# Autodesk Inventor assembly: Gantry Table With Chucks - V2
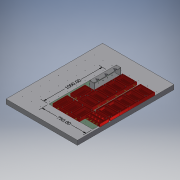
[picture p0: Inventor's stored thumbnail of the model, 180x180]
Saved by Autodesk Inventor 2019.4 (Build 234330000, 330)
## iProperties
Created: 2021-03-04
Part Number: Gantry Table With Chucks - V2
Document SubType Name: Assembly
Designer: caleb
Author: caleb
## Documents named in this file (6)
- C:\Users\cfang\Desktop\nebraska-silicon-lab\Hardware\ETL\Module Assembly\Gantry Table With Chucks - V2.iam
- C:\Users\cfang\Desktop\nebraska-silicon-lab\Hardware\ETL\Module Assembly\Gantry Base.ipt
- C:\Users\cfang\Desktop\nebraska-silicon-lab\Hardware\ETL\Module Assembly\Chuck - V2\Chuck - V2.ipt
- C:\Users\cfang\Desktop\nebraska-silicon-lab\Hardware\General Gantry\Gantry Tool Rack\Tool Rack Assembly.iam
- C:\Users\cfang\Desktop\nebraska-silicon-lab\Hardware\ETL\Module Assembly\Chuck - V2\Chuck - V2.iam
- C:\Users\cfang\Desktop\nebraska-silicon-lab\Hardware\ETL\Module Assembly\Chuck - Octopocket\Chuck - Octopocket.iam
## Components (18 placed, 4 different names)
1. Gantry Base:1 — Mate:14, Angle:9, Mate:15, Angle:10, Insert:1, Mate:16, Angle:11, Insert:2, Mate:17, Mate:18, Mate:19, Angle:12, Angle:13, Insert:4, Mate:20, Mate:21, Angle:14, Angle:15, Insert:5, Insert:6, Insert:7, Insert:8
2. Chuck - V2:7
3. Tool Rack Assembly:1 [sub-assembly] — Mate:14, Angle:9
4. Chuck - Octopocket:1 [sub-assembly] — Mate:17, Insert:7
5. Chuck - V2:24 [sub-assembly] — Mate:18, Angle:12, Insert:8
6. Chuck - V2:25 [sub-assembly] — Mate:19, Angle:13, Insert:4
7. Chuck - V2:26 [sub-assembly] — Mate:21, Angle:15, Insert:5
8. Chuck - V2:27 [sub-assembly] — Mate:20, Angle:14, Insert:6
9. Chuck - V2:13 [sub-assembly] — Mate:15, Angle:10, Insert:1
10. Chuck - V2:14 [sub-assembly]
11. Chuck - V2:15 [sub-assembly]
12. Chuck - V2:16 [sub-assembly]
13. Chuck - V2:17 [sub-assembly]
14. Chuck - V2:19 [sub-assembly] — Mate:16, Angle:11, Insert:2
15. Chuck - V2:20 [sub-assembly]
16. Chuck - V2:21 [sub-assembly]
17. Chuck - V2:22 [sub-assembly]
18. Chuck - V2:23 [sub-assembly]
## Component patterns: (5 elements, first: Chuck - V2:13), (5 elements, first: Chuck - V2:19)
## Relationships (22: Mate 8, Angle 7, Insert 7)
- Mate:14: Gantry Base:1 ↔ Tool Rack Assembly:1
- Angle:9 (0 deg): Gantry Base:1 ↔ Tool Rack Assembly:1
- Mate:15: Gantry Base:1 ↔ Chuck - V2:13
- Angle:10 (0 deg): Gantry Base:1 ↔ Chuck - V2:13
- Insert:1: Gantry Base:1 ↔ Chuck - V2:13
- Mate:16: Gantry Base:1 ↔ Chuck - V2:19
- Angle:11 (0 deg): Gantry Base:1 ↔ Chuck - V2:19
- Insert:2: Gantry Base:1 ↔ Chuck - V2:19
- Mate:17: Gantry Base:1 ↔ Chuck - Octopocket:1
- Mate:18: Gantry Base:1 ↔ Chuck - V2:24
- Mate:19: Gantry Base:1 ↔ Chuck - V2:25
- Angle:12 (0 deg): Gantry Base:1 ↔ Chuck - V2:24
- Angle:13 (0 deg): Gantry Base:1 ↔ Chuck - V2:25
- Insert:4: Gantry Base:1 ↔ Chuck - V2:25
- Mate:20: Gantry Base:1 ↔ Chuck - V2:27
- Mate:21: Gantry Base:1 ↔ Chuck - V2:26
- Angle:14 (180 deg): Gantry Base:1 ↔ Chuck - V2:27
- Angle:15 (0 deg): Gantry Base:1 ↔ Chuck - V2:26
- Insert:5: Gantry Base:1 ↔ Chuck - V2:26
- Insert:6: Gantry Base:1 ↔ Chuck - V2:27
- Insert:7: Gantry Base:1 ↔ Chuck - Octopocket:1
- Insert:8: Gantry Base:1 ↔ Chuck - V2:24
